# Autodesk Inventor assembly: wszystko
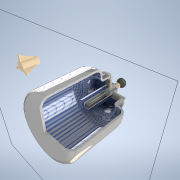
[picture p0: Inventor's stored thumbnail of the model, 180x180]
Saved by Autodesk Inventor 2021 (Build 250183000, 183)
## iProperties
Created: 2021-05-20
Part Number: wszystko
Document SubType Name: Assembly
Designer: Wojciech Wołczek
Author: Wojciech Wołczek
## Documents named in this file (11)
- D:\OneDrive\Documents\studia\I rok\labolatoria pracowni fizycznej\pracownia fizyczna 2021 xD\cw 25\wszystko.iam
- D:\OneDrive\Documents\studia\I rok\labolatoria pracowni fizycznej\pracownia fizyczna 2021 xD\cw 25\garnek.ipt
- D:\OneDrive\Documents\studia\I rok\labolatoria pracowni fizycznej\pracownia fizyczna 2021 xD\cw 25\dekiel.ipt
- D:\OneDrive\Documents\studia\I rok\labolatoria pracowni fizycznej\pracownia fizyczna 2021 xD\cw 25\dekieltop.ipt
- D:\OneDrive\Documents\studia\I rok\labolatoria pracowni fizycznej\pracownia fizyczna 2021 xD\cw 25\uchwyt1.ipt
- D:\OneDrive\Documents\studia\I rok\labolatoria pracowni fizycznej\pracownia fizyczna 2021 xD\cw 25\fiolka.ipt
- D:\OneDrive\Documents\studia\I rok\labolatoria pracowni fizycznej\pracownia fizyczna 2021 xD\cw 25\korek.ipt
- D:\OneDrive\Documents\studia\I rok\labolatoria pracowni fizycznej\pracownia fizyczna 2021 xD\cw 25\trmometr.iam
- D:\OneDrive\Documents\studia\I rok\labolatoria pracowni fizycznej\pracownia fizyczna 2021 xD\cw 25\stojak.ipt
- D:\OneDrive\Documents\studia\I rok\labolatoria pracowni fizycznej\pracownia fizyczna 2021 xD\cw 25\wodaxD.ipt
- D:\OneDrive\Documents\studia\I rok\labolatoria pracowni fizycznej\pracownia fizyczna 2021 xD\cw 25\ciecznnieznana.ipt
## Components (10 placed, 10 different names)
1. garnek:1 — Równoległe:1, Zestawiające:1, Równoległe:2, Równoległe:8, Równoległe:9, Równoległe:10
2. dekiel:1 — Równoległe:1, Zestawiające:1, Równoległe:2, Równoległe:3, Równoległe:4
3. dekieltop:1 — Równoległe:3, Równoległe:4, Równoległe:5
4. uchwyt1:1 — Równoległe:5, Walcowe:1, Zestawiające:2
5. fiolka:1 — Walcowe:1, Zestawiające:2, Równoległe:6, Równoległe:7, Równoległe:11, Równoległe:12
6. korek:1 — Równoległe:6, Równoległe:7, Zestawiające:3, Zestawiające:4
7. trmometr:1 [sub-assembly] — Zestawiające:3, Zestawiające:4, Kątowe:1
8. stojak:1 — Równoległe:8
9. wodaxD:1 — Równoległe:9, Równoległe:10
10. ciecznnieznana:1 — Równoległe:11, Równoległe:12
## Relationships (19: Flush 13, Mate 4, CylindricalJoint 1, Angle 1)
- Równoległe:1 [Flush]: garnek:1 ↔ dekiel:1
- Zestawiające:1 [Mate]: garnek:1 ↔ dekiel:1
- Równoległe:2 [Flush]: garnek:1 ↔ dekiel:1
- Równoległe:3 [Flush]: dekiel:1 ↔ dekieltop:1
- Równoległe:4 [Flush]: dekiel:1 ↔ dekieltop:1
- Równoległe:5 [Flush]: dekieltop:1 ↔ uchwyt1:1
- Walcowe:1 [CylindricalJoint]: uchwyt1:1 ↔ fiolka:1
- Zestawiające:2 [Mate]: uchwyt1:1 ↔ fiolka:1
- Równoległe:6 [Flush]: fiolka:1 ↔ korek:1
- Równoległe:7 [Flush]: fiolka:1 ↔ korek:1
- Zestawiające:3 [Mate]: korek:1 ↔ trmometr:1
- Zestawiające:4 [Mate]: korek:1 ↔ trmometr:1
- Równoległe:8 [Flush]: garnek:1 ↔ stojak:1
- Równoległe:9 [Flush]: garnek:1 ↔ wodaxD:1
- Równoległe:10 [Flush]: garnek:1 ↔ wodaxD:1
- Równoległe:11 [Flush]: fiolka:1 ↔ ciecznnieznana:1
- Równoległe:12 [Flush] (-40 mm): fiolka:1 ↔ ciecznnieznana:1
- Równoległe:13 [Flush] (381 mm)
- Kątowe:1 [Angle] (315 deg): trmometr:1
